# Autodesk Inventor assembly: arm
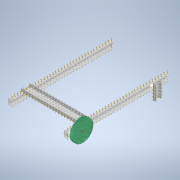
[picture p0: Inventor's stored thumbnail of the model, 180x180]
Saved by Autodesk Inventor 2020 (Build 240168000, 168)
## iProperties
Created: 2019-10-24
Part Number: arm
Document SubType Name: Assembly
Designer: Alex Zaccardelli
Author: Alex Zaccardelli
## Documents named in this file (8)
- D:\TrayBot Project\arm.iam
- D:\TrayBot Project\SIGBotsCADLibrary-20191023T040826Z-001\SIGBotsCADLibrary\SIGBotsCADLibrary\Structure\C-Channel 2 x 35 (aluminum).ipt
- D:\TrayBot Project\SIGBotsCADLibrary-20191023T040826Z-001\SIGBotsCADLibrary\SIGBotsCADLibrary\Motion\Gear HS 84 tooth (fixed).iam
- D:\TrayBot Project\SIGBotsCADLibrary-20191023T040826Z-001\SIGBotsCADLibrary\SIGBotsCADLibrary\Motion\Spacer 1.0 unit.ipt
- D:\TrayBot Project\SIGBotsCADLibrary-20191023T040826Z-001\SIGBotsCADLibrary\SIGBotsCADLibrary\Motion\Spacer 0.25 unit.ipt
- D:\TrayBot Project\SIGBotsCADLibrary-20191023T040826Z-001\SIGBotsCADLibrary\SIGBotsCADLibrary\Structure\C-Channel 3 x 16 (aluminum).ipt
- D:\TrayBot Project\SIGBotsCADLibrary-20191023T040826Z-001\SIGBotsCADLibrary\SIGBotsCADLibrary\Motion\Lock Plate.ipt
- D:\TrayBot Project\SIGBotsCADLibrary-20191023T040826Z-001\SIGBotsCADLibrary\SIGBotsCADLibrary\Structure\C-Channel 2 x 5 (aluminum).ipt
## Components (14 placed, 7 different names)
1. C-Channel 2 x 35 (aluminum):1 — Mate:3, Mate:4, Mate:8, Mate:11, Mate:12, Mate:16, Mate:17, Mate:18, Mate:22, Mate:23, Mate:24, Mate:25, Mate:26, Mate:27, Mate:28, Mate:29, Mate:30, Mate:31
2. Gear HS 84 tooth (fixed):1 [sub-assembly] — Mate:13, Mate:14, Mate:15
3. Spacer 1.0 unit:1 — Mate:1, Mate:2, Mate:3, Mate:4
4. Spacer 0.25 unit:1 — Mate:1, Mate:2, Mate:15
5. Spacer 1.0 unit:2 — Mate:8, Mate:13, Mate:14
6. Spacer 1.0 unit:3 — Mate:12
7. Spacer 0.25 unit:3 — Mate:11
8. C-Channel 3 x 16 (aluminum):1 — Mate:16, Mate:17, Mate:18, Mate:19, Mate:20, Mate:21
9. C-Channel 2 x 35 (aluminum):2 — Mate:19, Mate:20, Mate:21
10. Lock Plate:1 — Mate:22, Mate:23, Mate:24
11. Lock Plate:2 — Mate:25, Mate:26, Mate:27
12. C-Channel 2 x 5 (aluminum):1 — Mate:32, Mate:33, Mate:34
13. Spacer 1.0 unit:4 — Mate:28, Mate:29, Mate:32, Mate:33
14. Spacer 1.0 unit:5 — Mate:30, Mate:31, Mate:34
## Relationships (31: Mate 31)
- Mate:1: Spacer 1.0 unit:1 ↔ Spacer 0.25 unit:1
- Mate:2: Spacer 1.0 unit:1 ↔ Spacer 0.25 unit:1
- Mate:3: C-Channel 2 x 35 (aluminum):1 ↔ Spacer 1.0 unit:1
- Mate:4: C-Channel 2 x 35 (aluminum):1 ↔ Spacer 1.0 unit:1
- Mate:8: C-Channel 2 x 35 (aluminum):1 ↔ Spacer 1.0 unit:2
- [Mate]: Spacer 1.0 unit:3 ↔ Spacer 0.25 unit:3
- [Mate]: Spacer 1.0 unit:3 ↔ Spacer 0.25 unit:3
- Mate:11: C-Channel 2 x 35 (aluminum):1 ↔ Spacer 0.25 unit:3
- Mate:12: C-Channel 2 x 35 (aluminum):1 ↔ Spacer 1.0 unit:3
- Mate:13: Gear HS 84 tooth (fixed):1 ↔ Spacer 1.0 unit:2
- Mate:14: Gear HS 84 tooth (fixed):1 ↔ Spacer 1.0 unit:2
- Mate:15: Gear HS 84 tooth (fixed):1 ↔ Spacer 0.25 unit:1
- Mate:16: C-Channel 2 x 35 (aluminum):1 ↔ C-Channel 3 x 16 (aluminum):1
- Mate:17: C-Channel 2 x 35 (aluminum):1 ↔ C-Channel 3 x 16 (aluminum):1
- Mate:18: C-Channel 2 x 35 (aluminum):1 ↔ C-Channel 3 x 16 (aluminum):1
- Mate:19: C-Channel 3 x 16 (aluminum):1 ↔ C-Channel 2 x 35 (aluminum):2
- Mate:20: C-Channel 3 x 16 (aluminum):1 ↔ C-Channel 2 x 35 (aluminum):2
- Mate:21: C-Channel 3 x 16 (aluminum):1 ↔ C-Channel 2 x 35 (aluminum):2
- Mate:22: C-Channel 2 x 35 (aluminum):1 ↔ Lock Plate:1
- Mate:23: C-Channel 2 x 35 (aluminum):1 ↔ Lock Plate:1
- Mate:24: C-Channel 2 x 35 (aluminum):1 ↔ Lock Plate:1
- Mate:25: C-Channel 2 x 35 (aluminum):1 ↔ Lock Plate:2
- Mate:26: C-Channel 2 x 35 (aluminum):1 ↔ Lock Plate:2
- Mate:27: C-Channel 2 x 35 (aluminum):1 ↔ Lock Plate:2
- Mate:28: C-Channel 2 x 35 (aluminum):1 ↔ Spacer 1.0 unit:4
- Mate:29: C-Channel 2 x 35 (aluminum):1 ↔ Spacer 1.0 unit:4
- Mate:30: C-Channel 2 x 35 (aluminum):1 ↔ Spacer 1.0 unit:5
- Mate:31: C-Channel 2 x 35 (aluminum):1 ↔ Spacer 1.0 unit:5
- Mate:32: C-Channel 2 x 5 (aluminum):1 ↔ Spacer 1.0 unit:4
- Mate:33: C-Channel 2 x 5 (aluminum):1 ↔ Spacer 1.0 unit:4
- Mate:34: C-Channel 2 x 5 (aluminum):1 ↔ Spacer 1.0 unit:5
## Named parameters: d8_d0 = 0 mm, d9_d1 = 0 mm
